# Autodesk Inventor assembly: wheel
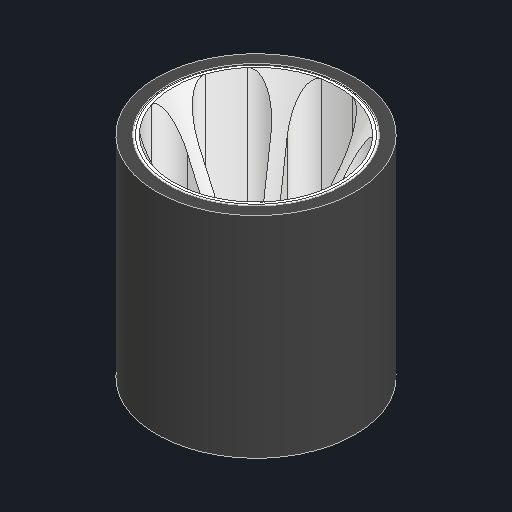
[picture p0: Inventor's stored thumbnail of the model, 512x512]
Saved by Autodesk Inventor 2023 (Build 270158000, 158)
## iProperties
Created: 2024-06-08
Part Number: wheel
Document SubType Name: Assembly
Designer: szymo
Mass: 47.0906 g
Surface Area: 368.378 cm^2
Volume: 47.3043 cm^3
Density: 0.995481 g/cm^3
TOTAL MASS: 0.0
Author: szymo
## Documents named in this file (3)
- D:\roboilo\robots\codename wafel - australia\3d_parts\rev4\wheel.iam
- D:\roboilo\robots\codename wafel - australia\3d_parts\rev4\felga.ipt
- D:\roboilo\robots\codename wafel - australia\3d_parts\rev4\oponka.ipt
## Components (2 placed, 2 different names)
1. felga:1 — Flush:1
2. oponka:1 — Flush:1
## Relationships (1: Flush 1)
- Flush:1: felga:1 ↔ oponka:1
